# Autodesk Inventor assembly: leg_assembly
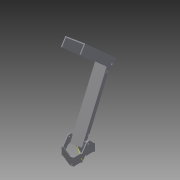
[picture p0: Inventor's stored thumbnail of the model, 180x180]
Saved by Autodesk Inventor 2015 (Build 190159000, 159)
## iProperties
Created: 2014-06-09
Part Number: leg_assembly
Document SubType Name: Assembly
Designer: L
Author: L
## Documents named in this file (5)
- C:\Users\Jaden\Documents\GitHub\SolidModels\stag_v2_01_pre_alpha\leg_assembly.iam
- C:\Users\Jaden\Documents\GitHub\SolidModels\stag_v2_01_pre_alpha\shoulder_servo_joint.ipt
- C:\Users\Jaden\Documents\GitHub\SolidModels\stag_v2_01_pre_alpha\upper_leg.iam
- C:\Users\Jaden\Documents\GitHub\SolidModels\stag_v2_01_pre_alpha\lower_leg.ipt
- C:\Users\Jaden\Documents\GitHub\SolidModels\stag_v2_01_pre_alpha\ServoHornHolder.ipt
## Components (5 placed, 4 different names)
1. shoulder_servo_joint:1 — Mate:1, Mate:5, Mate:8, Flush:1, Mate:9, Flush:2, Mate:10
2. upper_leg:1 [sub-assembly] — Mate:1, Mate:3, Mate:4, Mate:6, Mate:7, Angle:1
3. lower_leg:1 — Mate:3, Mate:4
4. ServoHornHolder:1 — Mate:6, Mate:7, Mate:8, Flush:1, Angle:1
5. ServoHornHolder:2 — Mate:9, Flush:2, Mate:10
## Relationships (12: Mate 9, Flush 2, Angle 1)
- Mate:1: shoulder_servo_joint:1 ↔ upper_leg:1
- Mate:3: upper_leg:1 ↔ lower_leg:1
- Mate:4: upper_leg:1 ↔ lower_leg:1
- Mate:5: shoulder_servo_joint:1
- Mate:6: upper_leg:1 ↔ ServoHornHolder:1
- Mate:7: upper_leg:1 ↔ ServoHornHolder:1
- Mate:8: shoulder_servo_joint:1 ↔ ServoHornHolder:1
- Flush:1: shoulder_servo_joint:1 ↔ ServoHornHolder:1
- Mate:9: shoulder_servo_joint:1 ↔ ServoHornHolder:2
- Flush:2: shoulder_servo_joint:1 ↔ ServoHornHolder:2
- Mate:10: shoulder_servo_joint:1 ↔ ServoHornHolder:2
- Angle:1 (0 deg): upper_leg:1 ↔ ServoHornHolder:1
